# Autodesk Inventor assembly: Baseplate - Metric Holes
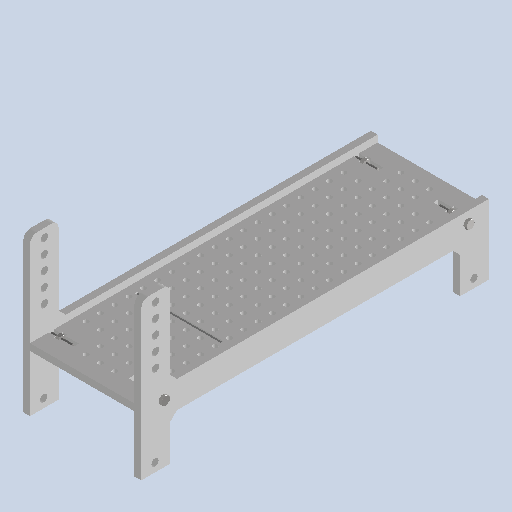
[picture p0: Inventor's stored thumbnail of the model, 512x512]
Saved by Autodesk Inventor 2022.1 (Build 261234000, 234)
## iProperties
Created: 2021-05-31
Part Number: Baseplate - Metric Holes
Document SubType Name: Assembly
Designer: John
Author: John
## Documents named in this file (5)
- C:\Users\owner\Desktop\Project 3 Modelling\Project 3 Autodesk Inventor Files\1. Baseplate\Baseplate - Metric Holes.iam
- C:\Users\owner\Desktop\Project 3 Modelling\Project 3 Autodesk Inventor Files\1. Baseplate\V3 Mounting Plate.ipt
- C:\Users\owner\Desktop\Project 3 Modelling\Project 3 Autodesk Inventor Files\1. Baseplate\V3 Mounting Wall.ipt
- C:\Users\owner\Desktop\Project 3 Modelling\Project 3 Autodesk Inventor Files\1. Baseplate\AS 1110 - M4 x 25.ipt
- C:\Users\owner\Desktop\Project 3 Modelling\Project 3 Autodesk Inventor Files\1. Baseplate\ISO 4032 - M4BS EN.ipt
## Components (11 placed, 4 different names)
1. V3 Mounting Plate:1 — Flush:1, Flush:2, Mate:1, Flush:3, Flush:5, Mate:5, Angle:1, Mate:9, Mate:13, Mate:17
2. V3 Mounting Wall:1 — Flush:1, Flush:2, Mate:1, Flush:4, Mate:3, Mate:4, Mate:14, Mate:15
3. V3 Mounting Wall:2 — Flush:3, Flush:4, Flush:5, Mate:6, Mate:7, Mate:10, Mate:11
4. AS 1110 - Metric M4 x 25:1 — Mate:10, Mate:11, Mate:12
5. AS 1110 - Metric M4 x 25:2 — Mate:6, Mate:7, Mate:8
6. AS 1110 - Metric M4 x 25:3 — Mate:2, Mate:3, Mate:4
7. AS 1110 - Metric M4 x 25:4 — Mate:14, Mate:15, Mate:16
8. BS EN 24032 - Metric M4:1 — Mate:12, Mate:13
9. BS EN 24032 - Metric M4:2 — Mate:8, Mate:9
10. BS EN 24032 - Metric M4:3 — Mate:2, Mate:5, Angle:1
11. BS EN 24032 - Metric M4:4 — Mate:16, Mate:17
## Relationships (23: Mate 17, Flush 5, Angle 1)
- Flush:1: V3 Mounting Plate:1 ↔ V3 Mounting Wall:1
- Flush:2: V3 Mounting Plate:1 ↔ V3 Mounting Wall:1
- Mate:1: V3 Mounting Plate:1 ↔ V3 Mounting Wall:1
- Flush:3: V3 Mounting Plate:1 ↔ V3 Mounting Wall:2
- Flush:4: V3 Mounting Wall:1 ↔ V3 Mounting Wall:2
- Flush:5: V3 Mounting Plate:1 ↔ V3 Mounting Wall:2
- Mate:2: AS 1110 - Metric M4 x 25:3 ↔ BS EN 24032 - Metric M4:3
- Mate:3: V3 Mounting Wall:1 ↔ AS 1110 - Metric M4 x 25:3
- Mate:4: V3 Mounting Wall:1 ↔ AS 1110 - Metric M4 x 25:3
- Mate:5: V3 Mounting Plate:1 ↔ BS EN 24032 - Metric M4:3
- Angle:1 (0 deg): V3 Mounting Plate:1 ↔ BS EN 24032 - Metric M4:3
- Mate:6: V3 Mounting Wall:2 ↔ AS 1110 - Metric M4 x 25:2
- Mate:7: V3 Mounting Wall:2 ↔ AS 1110 - Metric M4 x 25:2
- Mate:8: AS 1110 - Metric M4 x 25:2 ↔ BS EN 24032 - Metric M4:2
- Mate:9: V3 Mounting Plate:1 ↔ BS EN 24032 - Metric M4:2
- Mate:10: V3 Mounting Wall:2 ↔ AS 1110 - Metric M4 x 25:1
- Mate:11: V3 Mounting Wall:2 ↔ AS 1110 - Metric M4 x 25:1
- Mate:12: AS 1110 - Metric M4 x 25:1 ↔ BS EN 24032 - Metric M4:1
- Mate:13: V3 Mounting Plate:1 ↔ BS EN 24032 - Metric M4:1
- Mate:14: V3 Mounting Wall:1 ↔ AS 1110 - Metric M4 x 25:4
- Mate:15: V3 Mounting Wall:1 ↔ AS 1110 - Metric M4 x 25:4
- Mate:16: AS 1110 - Metric M4 x 25:4 ↔ BS EN 24032 - Metric M4:4
- Mate:17: V3 Mounting Plate:1 ↔ BS EN 24032 - Metric M4:4
